# Autodesk Inventor assembly: Pen Assembly
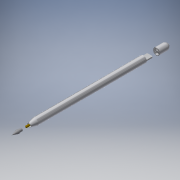
[picture p0: Inventor's stored thumbnail of the model, 180x180]
Saved by Autodesk Inventor 2018 (Build 220112000, 112)
## iProperties
Created: 2020-01-09
Part Number: Pen Assembly
Document SubType Name: Assembly
Designer: AOFUser
Author: AOFUser
## Documents named in this file (4)
- C:\Users\AOFUser\Desktop\Park_CAD\Class Project\Apple Pencil\Pen Assembly.iam
- C:\Users\AOFUser\Desktop\Park_CAD\Class Project\Apple Pencil\Pencil Body.ipt
- C:\Users\AOFUser\Desktop\Park_CAD\Class Project\Apple Pencil\Pencil Cab.ipt
- C:\Users\AOFUser\Desktop\Park_CAD\Class Project\Apple Pencil\Pencil Tip.ipt
## Components (3 placed, 3 different names)
1. Pencil Body:1 — Mate:1, Mate:2
2. Pencil Cab:1 — Mate:2
3. Pencil Tip:1 — Mate:1
## Relationships (2: Mate 2)
- Mate:1: Pencil Body:1 ↔ Pencil Tip:1
- Mate:2: Pencil Body:1 ↔ Pencil Cab:1
